# Autodesk Inventor assembly: Wheel Assembly
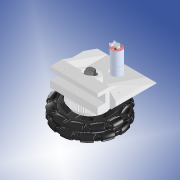
[picture p0: Inventor's stored thumbnail of the model, 180x180]
Saved by Autodesk Inventor 2017 SP1 (Build 210196100, 196)
## iProperties
Created: 2017-08-01
Part Number: Wheel Assembly
Document SubType Name: Assembly
Designer: Zach
Author: Zach
## Documents named in this file (10)
- C:\Users\Zach\Documents\GitHub\cr-laundry-robot\src\Base\Wheel Assembly\Wheel Assembly.iam
- C:\Users\Zach\Documents\GitHub\cr-laundry-robot\lib\Omni Wheel 6in\217-2585.ipt
- C:\Users\Zach\Documents\GitHub\cr-laundry-robot\lib\28x12x8mm Bearing.ipt
- C:\Users\Zach\Documents\GitHub\cr-laundry-robot\src\Base\Wheel Assembly\WA004.ipt
- C:\Users\Zach\Documents\GitHub\cr-laundry-robot\lib\DC Motor with Encoder\Motor.ipt
- C:\Users\Zach\Documents\GitHub\cr-laundry-robot\src\Base\Wheel Assembly\Wheel Assembly\Design Accelerator\Spur Gears1.iam
- C:\Users\Zach\Documents\GitHub\cr-laundry-robot\src\Base\Wheel Assembly\WA002.ipt
- C:\Users\Zach\Documents\GitHub\cr-laundry-robot\lib\AS 1110 - M12 x 100.ipt
- C:\Users\Zach\Documents\GitHub\cr-laundry-robot\lib\ISO 4032 - M12 - ISO.ipt
- C:\Users\Zach\Documents\GitHub\cr-laundry-robot\src\Base\Wheel Assembly\WA005.ipt
## Components (12 placed, 9 different names)
1. 217-2585:1 — Mate:1, Flush:1, Mate:2, Flush:2, Mate:27, Mate:28, Mate:34
2. 28x12x8mm Bearing:1 — Mate:1, Flush:1, Mate:32
3. 28x12x8mm Bearing:2 — Mate:2, Flush:2, Mate:43, Mate:44, Mate:47
4. WA004:1 — Mate:14, Mate:15, Mate:16, Mate:17, Mate:18, Mate:19, Mate:20, Mate:34, Mate:35, Mate:42, Mate:53, Mate:55, Mate:57
5. Motor:1 — Mate:14, Mate:15, Mate:16, Mate:54, Mate:56
6. 28x12x8mm Bearing:3 — Mate:19, Mate:20
7. 28x12x8mm Bearing:4 — Mate:17, Mate:18, Mate:46
8. Spur Gears:1 [sub-assembly] — Mate:27, Mate:28, Mate:35, Mate:53, Mate:54, Mate:55, Mate:58
9. WA002:1 — Mate:32, Mate:47
10. AS 1110 - Metric M12 x 100:1 — Mate:43, Mate:44, Mate:45, Mate:51, Mate:52
11. ISO 4032 M12:1 — Mate:45, Mate:46
12. WA005:1 — Mate:56, Mate:57, Mate:58
## Relationships (30: Mate 28, Flush 2)
- Mate:1: 217-2585:1 ↔ 28x12x8mm Bearing:1
- Flush:1: 217-2585:1 ↔ 28x12x8mm Bearing:1
- Mate:2: 217-2585:1 ↔ 28x12x8mm Bearing:2
- Flush:2: 217-2585:1 ↔ 28x12x8mm Bearing:2
- Mate:14: WA004:1 ↔ Motor:1
- Mate:15: WA004:1 ↔ Motor:1
- Mate:16: WA004:1 ↔ Motor:1
- Mate:17: WA004:1 ↔ 28x12x8mm Bearing:4
- Mate:18: WA004:1 ↔ 28x12x8mm Bearing:4
- Mate:19: WA004:1 ↔ 28x12x8mm Bearing:3
- Mate:20: WA004:1 ↔ 28x12x8mm Bearing:3
- Mate:27: 217-2585:1 ↔ Spur Gears:1
- Mate:28: 217-2585:1 ↔ Spur Gears:1
- Mate:32: 28x12x8mm Bearing:1 ↔ WA002:1
- Mate:34: 217-2585:1 ↔ WA004:1
- Mate:35: WA004:1 ↔ Spur Gears:1
- Mate:42: WA004:1
- Mate:43: 28x12x8mm Bearing:2 ↔ AS 1110 - Metric M12 x 100:1
- Mate:44: 28x12x8mm Bearing:2 ↔ AS 1110 - Metric M12 x 100:1
- Mate:45: AS 1110 - Metric M12 x 100:1 ↔ ISO 4032 M12:1
- Mate:46: 28x12x8mm Bearing:4 ↔ ISO 4032 M12:1
- Mate:47: 28x12x8mm Bearing:2 ↔ WA002:1
- Mate:51: AS 1110 - Metric M12 x 100:1
- Mate:52: AS 1110 - Metric M12 x 100:1
- Mate:53: WA004:1 ↔ Spur Gears:1
- Mate:54: Motor:1 ↔ Spur Gears:1
- Mate:55: WA004:1 ↔ Spur Gears:1
- Mate:56: Motor:1 ↔ WA005:1
- Mate:57: WA004:1 ↔ WA005:1
- Mate:58: Spur Gears:1 ↔ WA005:1
